# Autodesk Inventor assembly: CJ2D16-200Z(0_1_0)
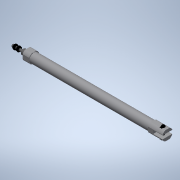
[picture p0: Inventor's stored thumbnail of the model, 180x180]
Saved by Autodesk Inventor 2022.3 (Build 263350000, 350)
## iProperties
Created: 2020-02-05
Part Number: CJ2D16-200Z(0_1_0)
Catalog Web Link: www.cadenas.de
Description: CJ2-Z/CDJ2-Z-Air Cylinder/Standard: Double Acting Single Rod
Vendor: SMC
Document SubType Name: Assembly
Designer: psadmin
Manufacturer: SMC
Category: PARTsolutions
Company: SMC
PSOL_IDENT_0: {$CADENAS_DATA\23d-libs\smc_jp\actuator\standard_air_cylinder\cj2\cj2_z_asmtab.prj},309 {VTYP=3D},{S
PSOL_IDENT_1: TYP=ASSTAB},{NB=CJ2D16-200Z(0_1_0)},{LINA=CJ2D16-200Z},{NN=CJ2-Z/CDJ2-Z},{DATE=19.12.2019 04:36:36},
PSOL_IDENT_2: {GEOMDATE=13.04.2018 02:47:55},{VERSION=},{LINEID=430},{WBVAR=MAGNET,AUTOSWITCH,LEAD,NUMBER,CUSHION,
PSOL_IDENT_3: STROKE,POS,PORT,STOP,BRACKET,RODB,MOUNTING,OMSC,OMSCXC3,OMSCXC51,THREAD},{WBNUMERIC=STROKE,POS}  {NB=
PSOL_IDENT_4: CJ2D16-200Z(0_1_0)},{LINA=CJ2D16-200Z},{KT=DUMMY},{NENN=CJ2D16-200Z},{ORDER=CJ2D16-200Z},{BORE=16},{
PSOL_IDENT_5: MOUNT=(D) Double clevis},{MOUNTX=D},{MAGNET=},{AUTOSWITCH=},{AUTOSWX='','N/A'},{LEAD=},{LEADX= '','N
PSOL_IDENT_6: /A' },{NUMBER=},{CUSHION=},{CUSHIONX= '','(-) Rubber cushion','A','(A) Air cushion' },{SWSIGNX= '','
PSOL_IDENT_7: N/A' },{STROKE=200},{STDSTROKE=15,30,45,60,75,100,125,150,175,200},{STROKE1X=[1:400/1]},{SMIN=1},{SM
PSOL_IDENT_8: INASW1=10},{SMINASW2=15},{SMAX1=400},{POS=0},{PORT=},{STOP=1},{COM=Please confirm the conditions of
PSOL_IDENT_9: use with SMC},{BRACKET=},{RODB=},{RODBX= '', '(-) None', 'V', '(V) Single knuckle joint', 'W'  , '(W
PSOL_IDENT_10: ) Double knuckle joint', 'T', '(T) Rod end cap (Flat type)', 'U'  , '(U) Rod end cap (Round type)' }
PSOL_IDENT_11: ,{MOUNTING=},{OMSC=},{OMSCXC3=},{OMSCXC51=},{THREAD=0},{MOUNTINGX='','N/A'},{BRACKETX='','(-) None','
PSOL_IDENT_12: N','(N) Pivot bracket is shipped together with the product,but not assembled.'},{PORTX='', '(-) Perp
PSOL_IDENT_13: endicular to axis'},{SW=B},{OMSCX= '','(-) None','-XB6','(XB6) Heat resistant cylinder (-10 to 150 d
PSOL_IDENT_14: egree Celsius)','-XB7','(XB7) Cold resistant cylinder (-40 to 70 degree Celsius)','-XB9','(XB9) Low
PSOL_IDENT_15: speed cylinder (10 to 50 mm/s)','-XC22','(XC22) Fluororubber seals','-XC85','(XC85) Grease specifica
PSOL_IDENT_16: tion for food processing machines', '-X446'  , '(X446) PTFE grease' },{A=2.5},{XC3= '','(-) None','-
PSOL_IDENT_17: XC3AB','(XC3AB) Rod port location viewed: A,Head port location viewed: B','-XC3AC','(XC3AC) Rod port
PSOL_IDENT_18: location viewed: A,Head port location viewed: C','-XC3AD','(XC3AD) Rod port location viewed: A,Head
PSOL_IDENT_19: port location viewed: D','-XC3BA','(XC3BA) Rod port location viewed: B,Head port location viewed: A'
PSOL_IDENT_20: ,'-XC3BB','(XC3BB) Rod port location viewed: B,Head port location viewed: B','-XC3BC','(XC3BC) Rod p
PSOL_IDENT_21: ort location viewed: B,Head port location viewed: C','-XC3BD','(XC3BD) Rod port location viewed: B,H
PSOL_IDENT_22: ead port location viewed: D','-XC3CA','(XC3CA) Rod port location viewed: C,Head port location viewed
PSOL_IDENT_23: : A','-XC3CB','(XC3CB) Rod port location viewed: C,Head port location viewed: B','-XC3CC','(XC3CC) R
PSOL_IDENT_24: od port location viewed: C,Head port location viewed: C','-XC3CD','(XC3CD) Rod port location viewed:
PSOL_IDENT_25: C,Head port location viewed: D','-XC3DA','(XC3DA) Rod port location viewed: D,Head port location vi
PSOL_IDENT_26: ewed: A','-XC3DB','(XC3DB) Rod port location viewed: D,Head port location viewed: B','-XC3DC','(XC3D
PSOL_IDENT_27: C) Rod port location viewed: D,Head port location viewed: C','-XC3DD','(XC3DD) Rod port location vie
PSOL_IDENT_28: wed: D,Head port location viewed: D' },{XC51= '','(-) None','-XC51H4','(XC51H4) Hose nipple type: ø4
PSOL_IDENT_29: /2.5 with restriction','-XC51H6','(XC51H6) Hose nipple type: ø6/4 with restriction','-XC51MH4','(XC5
PSOL_IDENT_30: 1MH4) Hose nipple type: ø4/2.5 without restriction','-XC51MH6','(XC51MH6) Hose nipple type: ø6/4 wit
PSOL_IDENT_31: hout restriction' },{BMP=D},{PPATH=cj2_z/assembly/cj2_z_asmsbl.prj},{OMSCXX= '','(-) None','-XB6','(
PSOL_IDENT_32: XB6) Heat resistant cylinder (-10 to 150 degree Celsius)','-XB7','(XB7) Cold resistant cylinder (-40
PSOL_IDENT_33: to 70 degree Celsius)','-XB9','(XB9) Low speed cylinder (10 to 50 mm/s)','-XC22','(XC22) Fluororubb
PSOL_IDENT_34: er seals','-XC85','(XC85) Grease specification for food processing machines', '-X446'  , '(X446) PTF
PSOL_IDENT_35: E grease' ,'-X2838','(X2838) Double clevis (With one-touch connecting pin)' }
NN: CJ2-Z/CDJ2-Z
NT: Air Cylinder/Standard: Double Acting Single Rod
NB: CJ2D16-200Z(0_1_0)
NBSYN: $ORDER.($POS._$STOP._$THREAD.)
LINA: CJ2D16-200Z
BORE: 16
MOUNT: (D) Double clevis
MAGNET: (-) Without magnet
AUTOSWITCH: N/A
LEAD: N/A
NUMBER: N/A
CUSHION: (-) Rubber cushion
STROKE: 200
POS: 0
PORT: (-) Perpendicular to axis
STOP: Manufacturable stroke
BRACKET: (-) None
RODB: (-) None
MOUNTING: N/A
OMSC: (-) None
OMSCXC3: (-) None
OMSCXC51: (-) None
THREAD: on
SUPPLIER: SMC
ARTICLENO: CJ2D16-200Z(0_1_0)
BOMINFO: CJ2D16-200Z
CREATOR: CADENAS GmbH
Title: CJ2D16-200Z
Author: Cadenas PARTsolutions
Comments: Air Cylinder/Standard: Double Acting Single Rod
## Documents named in this file (5)
- C:\Users\YusukeKunita\Documents\GrabCAD\Development\BasicParts\AirCylinder\CJ2D16-200Z\CJ2D16-200Z.iam
- C:\Users\YusukeKunita\Documents\GrabCAD\Development\BasicParts\AirCylinder\CJ2D16-200Z\CJ2D16-200Z_BODY.ipt
- C:\Users\YusukeKunita\Documents\GrabCAD\Development\BasicParts\AirCylinder\CJ2D16-200Z\CJ2D16-200Z_ROD.ipt
- C:\Users\YusukeKunita\Documents\GrabCAD\Development\BasicParts\AirCylinder\CJ2D16-200Z\NTJ-015C.ipt
- C:\Users\YusukeKunita\Documents\GrabCAD\Development\BasicParts\AirCylinder\CJ2D16-200Z\CJ2-Z_CD-Z015.ipt
## Components (5 placed, 4 different names)
1. CJ2D16-200Z_BODY:1 — body_Z@1 <-> ROD_BODY_Z@2, body_YZ@1 <-> ROD_BODY_YZ@2, BODY_PIN_XY@1 <-> cd_XY@5, BODY_PIN_Z@1 <-> cd_Z@5, BODY_PIN_YZ@1 <-> cd_YZ@5
2. CJ2D16-200Z_ROD:1 — body_Z@1 <-> ROD_BODY_Z@2, body_YZ@1 <-> ROD_BODY_YZ@2, rodnt1_XY@2 <-> ntj_XY@3, rodnt1_Z@2 <-> ntj_Z@3, rodnt1_YZ@2 <-> ntj_YZ@3, rodnt1_XY@2 <-> ntj_XY@4, rodnt1_Z@2 <-> ntj_Z@4, rodnt1_YZ@2 <-> ntj_YZ@4
3. NTJ-015C:1 — rodnt1_XY@2 <-> ntj_XY@3, rodnt1_Z@2 <-> ntj_Z@3, rodnt1_YZ@2 <-> ntj_YZ@3
4. NTJ-015C:2 — rodnt1_XY@2 <-> ntj_XY@4, rodnt1_Z@2 <-> ntj_Z@4, rodnt1_YZ@2 <-> ntj_YZ@4
5. CJ2-Z_CD-Z015:1 — BODY_PIN_XY@1 <-> cd_XY@5, BODY_PIN_Z@1 <-> cd_Z@5, BODY_PIN_YZ@1 <-> cd_YZ@5
## Relationships (11: Mate 6, Angle 4, Flush 1)
- body_Z@1 <-> ROD_BODY_Z@2 [Mate]: CJ2D16-200Z_BODY:1 ↔ CJ2D16-200Z_ROD:1
- body_YZ@1 <-> ROD_BODY_YZ@2 [Angle] (0 deg): CJ2D16-200Z_BODY:1 ↔ CJ2D16-200Z_ROD:1
- rodnt1_XY@2 <-> ntj_XY@3 [Mate] (2.5 mm): CJ2D16-200Z_ROD:1 ↔ NTJ-015C:1
- rodnt1_Z@2 <-> ntj_Z@3 [Mate]: CJ2D16-200Z_ROD:1 ↔ NTJ-015C:1
- rodnt1_YZ@2 <-> ntj_YZ@3 [Angle] (0 deg): CJ2D16-200Z_ROD:1 ↔ NTJ-015C:1
- rodnt1_XY@2 <-> ntj_XY@4 [Flush]: CJ2D16-200Z_ROD:1 ↔ NTJ-015C:2
- rodnt1_Z@2 <-> ntj_Z@4 [Mate]: CJ2D16-200Z_ROD:1 ↔ NTJ-015C:2
- rodnt1_YZ@2 <-> ntj_YZ@4 [Angle] (0 deg): CJ2D16-200Z_ROD:1 ↔ NTJ-015C:2
- BODY_PIN_XY@1 <-> cd_XY@5 [Mate]: CJ2D16-200Z_BODY:1 ↔ CJ2-Z_CD-Z015:1
- BODY_PIN_Z@1 <-> cd_Z@5 [Mate]: CJ2D16-200Z_BODY:1 ↔ CJ2-Z_CD-Z015:1
- BODY_PIN_YZ@1 <-> cd_YZ@5 [Angle] (0 deg): CJ2D16-200Z_BODY:1 ↔ CJ2-Z_CD-Z015:1
